# Autodesk Inventor assembly: Mechanical Pencil
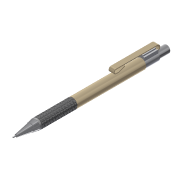
[picture p0: Inventor's stored thumbnail of the model, 180x180]
Saved by Autodesk Inventor 2022 (Build 260148000, 148)
## iProperties
Created: 2008-09-23
Part Number: Mechanical Pencil
Document SubType Name: Assembly
Designer: Mark Flayler
Mass: 17.7021 g
Surface Area: 137.125 cm^2
Volume: 3.92388 cm^3
Density: 4.51137 g/cm^3
Author: Mark Flayler
## Documents named in this file (16)
- C:\Autodesk Inventor 2022 Advanced Assembly Modeling Practice Files\Mechanical_Pencil_Assembly Tools\Mechanical Pencil.iam
- C:\Autodesk Inventor 2022 Advanced Assembly Modeling Practice Files\Mechanical_Pencil_Assembly Tools\Clip.ipt
- C:\Autodesk Inventor 2022 Advanced Assembly Modeling Practice Files\Mechanical_Pencil_Assembly Tools\Cone.ipt
- C:\Autodesk Inventor 2022 Advanced Assembly Modeling Practice Files\Mechanical_Pencil_Assembly Tools\Coupling.ipt
- C:\Autodesk Inventor 2022 Advanced Assembly Modeling Practice Files\Mechanical_Pencil_Assembly Tools\Dispenser Ring.ipt
- C:\Autodesk Inventor 2022 Advanced Assembly Modeling Practice Files\Mechanical_Pencil_Assembly Tools\Dispenser.ipt
- C:\Autodesk Inventor 2022 Advanced Assembly Modeling Practice Files\Mechanical_Pencil_Assembly Tools\Eraser Cap.ipt
- C:\Autodesk Inventor 2022 Advanced Assembly Modeling Practice Files\Mechanical_Pencil_Assembly Tools\Eraser.ipt
- C:\Autodesk Inventor 2022 Advanced Assembly Modeling Practice Files\Mechanical_Pencil_Assembly Tools\Lead Guide.ipt
- C:\Autodesk Inventor 2022 Advanced Assembly Modeling Practice Files\Mechanical_Pencil_Assembly Tools\Shaft Dispenser.ipt
- C:\Autodesk Inventor 2022 Advanced Assembly Modeling Practice Files\Mechanical_Pencil_Assembly Tools\Spring.ipt
- C:\Autodesk Inventor 2022 Advanced Assembly Modeling Practice Files\Mechanical_Pencil_Assembly Tools\Upper Shaft.ipt
- C:\Autodesk Inventor 2022 Advanced Assembly Modeling Practice Files\Mechanical_Pencil_Assembly Tools\Pencil Shaft.ipt
- C:\Autodesk Inventor 2022 Advanced Assembly Modeling Practice Files\Mechanical_Pencil_Assembly Tools\Sleeve.ipt
- C:\Autodesk Inventor 2022 Advanced Assembly Modeling Practice Files\Mechanical_Pencil_Assembly Tools\Grip.ipt
- C:\Autodesk Inventor 2022 Advanced Assembly Modeling Practice Files\Mechanical_Pencil_Assembly Tools\Ring.ipt
## Components (15 placed, 15 different names)
1. Pencil Shaft:1 — Insert:2, Insert:3, Insert:4
2. Clip:1 — Mate:1, Mate:2, Mate:3
3. Cone:1 — Insert:1, Insert:5, Insert:6, Insert:9
4. Coupling:1 — Insert:7
5. Dispenser Ring:1 — Insert:5
6. Dispenser:1 — Insert:6, Insert:7, Mate:4
7. Eraser Cap:1 — Insert:3
8. Eraser:1 — Insert:2
9. Lead Guide:1 — Insert:1
10. Shaft Dispenser:1 — Insert:9, Mate:5
11. Spring:1 — Mate:4, Mate:5
12. Upper Shaft:1 — Mate:1, Mate:2, Mate:3, Insert:4, Flush:1
13. Sleeve:1
14. Grip:1
15. Ring:1
## Relationships (19: Insert 11, Mate 7, Flush 1)
- Mate:1: Clip:1 ↔ Upper Shaft:1
- Mate:2: Clip:1 ↔ Upper Shaft:1
- Insert:1 (-1 mm): Cone:1 ↔ Lead Guide:1
- Insert:2: Pencil Shaft:1 ↔ Eraser:1
- Insert:3: Pencil Shaft:1 ↔ Eraser Cap:1
- Mate:3: Clip:1 ↔ Upper Shaft:1
- Insert:4 (4 mm): Pencil Shaft:1 ↔ Upper Shaft:1
- Insert:5: Cone:1 ↔ Dispenser Ring:1
- Insert:6: Cone:1 ↔ Dispenser:1
- Insert:7: Coupling:1 ↔ Dispenser:1
- [Insert]: Cone:1 ↔ Ring:1
- Mate:4: Dispenser:1 ↔ Spring:1
- Insert:9: Cone:1 ↔ Shaft Dispenser:1
- Mate:5: Shaft Dispenser:1 ↔ Spring:1
- [Mate]: Upper Shaft:1 ↔ Sleeve:1
- [Mate]: Upper Shaft:1 ↔ Sleeve:1
- Flush:1: Upper Shaft:1
- [Insert]: Sleeve:1 ↔ Grip:1
- [Insert]: Grip:1 ↔ Ring:1
